# Autodesk Inventor assembly: WheelAdapter-4mm
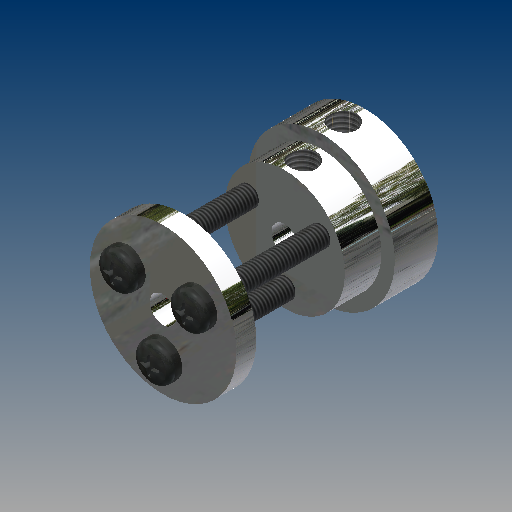
[picture p0: Inventor's stored thumbnail of the model, 512x512]
Saved by Autodesk Inventor 2017 (Build 210142000, 142)
## iProperties
Created: 2017-05-07
Part Number: WheelAdapter-4mm
Document SubType Name: Assembly
Designer: zallen
Catalog Web Link: https://www.pololu.com/product/2672
Author: zallen
## Documents named in this file (6)
- C:\Users\zallen\Documents\Autodesk Inventor Projects\Pololu\WheelAdapter-4mm\WheelAdapter-4mm.iam
- C:\Users\zallen\Documents\Autodesk Inventor Projects\Pololu\WheelAdapter-4mm\WheelAdapter-4mm-1.ipt
- C:\Users\zallen\Documents\Autodesk Inventor Projects\Pololu\WheelAdapter-4mm\WheelAdapter-4mm-2.ipt
- C:\Users\zallen\Documents\Autodesk Inventor Projects\Pololu\WheelAdapter-4mm\WheelAdapter-4mm\Design Accelerator\Bolted Connection1.iam
- C:\Users\zallen\Documents\Autodesk Inventor Projects\Pololu\WheelAdapter-4mm\WheelAdapter-4mm\Design Accelerator\Bolted Connection2.iam
- C:\Users\zallen\Documents\Autodesk Inventor Projects\Pololu\WheelAdapter-4mm\WheelAdapter-4mm\Design Accelerator\Bolted Connection3.iam
## Components (5 placed, 3 different names)
1. WheelAdapter-4mm-1:1 — Mate:1, Mate:2, Mate:3
2. WheelAdapter-4mm-2:1 — Flush:1, Mate:1, Mate:2, Mate:3, Mate:4, Mate:5, Mate:6, Mate:7, Mate:8, Mate:9
3. Bolted Connection:1 [sub-assembly] — Mate:4, Mate:5
4. Bolted Connection:2 [sub-assembly] — Mate:6, Mate:7
5. Bolted Connection:3 [sub-assembly] — Mate:8, Mate:9
## Relationships (10: Mate 9, Flush 1)
- Flush:1: WheelAdapter-4mm-2:1
- Mate:1: WheelAdapter-4mm-1:1 ↔ WheelAdapter-4mm-2:1
- Mate:2: WheelAdapter-4mm-1:1 ↔ WheelAdapter-4mm-2:1
- Mate:3: WheelAdapter-4mm-1:1 ↔ WheelAdapter-4mm-2:1
- Mate:4: WheelAdapter-4mm-2:1 ↔ Bolted Connection:1
- Mate:5: WheelAdapter-4mm-2:1 ↔ Bolted Connection:1
- Mate:6: WheelAdapter-4mm-2:1 ↔ Bolted Connection:2
- Mate:7: WheelAdapter-4mm-2:1 ↔ Bolted Connection:2
- Mate:8: WheelAdapter-4mm-2:1 ↔ Bolted Connection:3
- Mate:9: WheelAdapter-4mm-2:1 ↔ Bolted Connection:3
